# Autodesk Inventor assembly: DriveTrainPlateMecanum2017-18BackUp
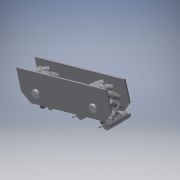
[picture p0: Inventor's stored thumbnail of the model, 180x180]
Saved by Autodesk Inventor 2017 (Build 210142000, 142)
## iProperties
Created: 2017-09-16
Part Number: DriveTrainPlateMecanum2017-18BackUp
Document SubType Name: Assembly
Designer: User
Author: User
## Documents named in this file (5)
- C:\Robotics\CAD\2017-18_CAD\DriveTrainMecanumDemo1.iam
- C:\Robotics\CAD\2017-18_CAD\MecanumDriveTrainPlate17-18.ipt
- C:\Robotics\CAD\2017-18_CAD\LeftDriveTrainMecanum2017-18.iam
- C:\Robotics\CAD\COTSParts\Motors\Andymark 2964  NeveRest 40 Motor.ipt
- C:\Robotics\CAD\2017-18_CAD\MecanumDriveTrainPlate17-18-NoMotor.ipt
## Components (6 placed, 4 different names)
1. LeftDriveTrainMecanum2017-18:1 [sub-assembly] — Mate:5, Mate:9, Mate:11, Mate:12
2. LeftDriveTrainMecanum2017-18:2 [sub-assembly] — Mate:6, Mate:7, Mate:10, Mate:13
3. MecanumDriveTrainPlate17-18:2 — Mate:5, Mate:6, Mate:7, Mate:9, Mate:12
4. Andymark 2964  NeveRest 40 Motor:1
5. Andymark 2964  NeveRest 40 Motor:2
6. MecanumDriveTrainPlate17-18-NoMotor:1 — Mate:10, Mate:11, Mate:13
## Relationships (8: Mate 8)
- Mate:5: LeftDriveTrainMecanum2017-18:1 ↔ MecanumDriveTrainPlate17-18:2
- Mate:6: LeftDriveTrainMecanum2017-18:2 ↔ MecanumDriveTrainPlate17-18:2
- Mate:7: LeftDriveTrainMecanum2017-18:2 ↔ MecanumDriveTrainPlate17-18:2
- Mate:9: LeftDriveTrainMecanum2017-18:1 ↔ MecanumDriveTrainPlate17-18:2
- Mate:10: LeftDriveTrainMecanum2017-18:2 ↔ MecanumDriveTrainPlate17-18-NoMotor:1
- Mate:11: LeftDriveTrainMecanum2017-18:1 ↔ MecanumDriveTrainPlate17-18-NoMotor:1
- Mate:12: LeftDriveTrainMecanum2017-18:1 ↔ MecanumDriveTrainPlate17-18:2
- Mate:13: LeftDriveTrainMecanum2017-18:2 ↔ MecanumDriveTrainPlate17-18-NoMotor:1
